# Autodesk Inventor assembly: ElectronicsHousing
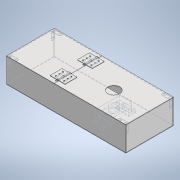
[picture p0: Inventor's stored thumbnail of the model, 180x180]
Saved by Autodesk Inventor 2020 (Build 240168000, 168)
## iProperties
Created: 2021-11-12
Part Number: ElectronicsHousing
Document SubType Name: Assembly
Designer: 17185
Author: 17185
## Documents named in this file (8)
- C:\Users\17185\Desktop\chassis draft\ElectronicsHousing\ElectronicsHousing.iam
- C:\Users\17185\Desktop\chassis draft\ElectronicsHousing\ElectronicsCasing.iam
- C:\Users\17185\Desktop\chassis draft\CornerBrace.ipt
- C:\Users\17185\Desktop\chassis draft\ElectronicsHousing\FixedPanel.ipt
- C:\Users\17185\Desktop\chassis draft\ElectronicsHousing\FreePanel.ipt
- C:\Users\17185\Desktop\chassis draft\Hinge\leaf.ipt
- C:\Users\17185\Desktop\chassis draft\Hinge\Pin.ipt
- C:\Users\17185\Desktop\chassis draft\arm standoff\arm standoff.iam
## Components (14 placed, 7 different names)
1. ElectronicsCasing:1 [sub-assembly] — Mate:1, Flush:6, Mate:2, Mate:3, Mate:4, Mate:5, Mate:6, Flush:7, Flush:8, Mate:17
2. FixedPanel:1 — Mate:7, Flush:7, Flush:8, Flush:9, Mate:16, Mate:18
3. FreePanel:1 — Flush:9, Mate:14, Mate:15, Mate:16
4. CornerBrace:1 — Flush:1, Flush:4, Mate:1, Flush:6, Mate:2
5. CornerBrace:2 — Flush:3, Flush:4, Mate:3
6. CornerBrace:3 — Flush:1, Flush:2, Flush:5, Mate:6, Mate:7
7. CornerBrace:4 — Flush:2, Flush:3, Flush:5, Mate:4, Mate:5
8. leaf:2 — Flush:14, Mate:12, Mate:14
9. leaf:3 — Flush:13, Mate:11
10. leaf:4 — Mate:10, Flush:11
11. Pin:1 — Flush:13, Mate:11, Mate:13, Flush:15
12. Pin:2 — Mate:10, Flush:11, Flush:14, Mate:12
13. leaf:5 — Mate:13, Flush:15, Mate:15
14. arm standoff:1 [sub-assembly] — Mate:17, Mate:18
## Relationships (29: Mate 16, Flush 13)
- Flush:1: CornerBrace:1 ↔ CornerBrace:3
- Flush:2: CornerBrace:3 ↔ CornerBrace:4
- Flush:3: CornerBrace:2 ↔ CornerBrace:4
- Flush:4: CornerBrace:1 ↔ CornerBrace:2
- Flush:5: CornerBrace:3 ↔ CornerBrace:4
- Mate:1: ElectronicsCasing:1 ↔ CornerBrace:1
- Flush:6: ElectronicsCasing:1 ↔ CornerBrace:1
- Mate:2: ElectronicsCasing:1 ↔ CornerBrace:1
- Mate:3: ElectronicsCasing:1 ↔ CornerBrace:2
- Mate:4: ElectronicsCasing:1 ↔ CornerBrace:4
- Mate:5: ElectronicsCasing:1 ↔ CornerBrace:4
- Mate:6: ElectronicsCasing:1 ↔ CornerBrace:3
- Mate:7: FixedPanel:1 ↔ CornerBrace:3
- Flush:7: ElectronicsCasing:1 ↔ FixedPanel:1
- Flush:8: ElectronicsCasing:1 ↔ FixedPanel:1
- Flush:9: FixedPanel:1 ↔ FreePanel:1
- Mate:10: leaf:4 ↔ Pin:2
- Flush:11: leaf:4 ↔ Pin:2
- Flush:13: leaf:3 ↔ Pin:1
- Flush:14: leaf:2 ↔ Pin:2
- Mate:11: leaf:3 ↔ Pin:1
- Mate:12: leaf:2 ↔ Pin:2
- Mate:13: Pin:1 ↔ leaf:5
- Flush:15: Pin:1 ↔ leaf:5
- Mate:14: FreePanel:1 ↔ leaf:2
- Mate:15: FreePanel:1 ↔ leaf:5
- Mate:16: FixedPanel:1 ↔ FreePanel:1
- Mate:17: ElectronicsCasing:1 ↔ arm standoff:1
- Mate:18: FixedPanel:1 ↔ arm standoff:1
